# Autodesk Inventor assembly: S2x1
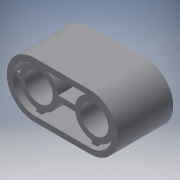
[picture p0: Inventor's stored thumbnail of the model, 180x180]
Saved by Autodesk Inventor 2019 (Build 230136000, 136)
## iProperties
Created: 2019-01-31
Part Number: S2x1
Document SubType Name: Assembly
Designer: Varga Daniel
Author: Varga Daniel
## Documents named in this file (2)
- C:\!_Dani\!_cloud\OneDrive\!_munka\Revolution\RevvyDemoKit\Structural parts\Straight Beams\S2x1.iam
- C:\!_Dani\!_cloud\OneDrive\!_munka\Revolution\RevvyDemoKit\Structural parts\Straight Beams\straight_beam_single_end_part.ipt
## Components (2 placed, 1 different names)
1. straight_beam_single_end_part:1 — Flush:1, Mate:1, Flush:2
2. straight_beam_single_end_part:2 — Flush:1, Mate:1, Flush:2
## Relationships (3: Flush 2, Mate 1)
- Flush:1: straight_beam_single_end_part:1 ↔ straight_beam_single_end_part:2
- Mate:1: straight_beam_single_end_part:1 ↔ straight_beam_single_end_part:2
- Flush:2: straight_beam_single_end_part:1 ↔ straight_beam_single_end_part:2
